# Autodesk Inventor assembly: Assey-N-N-body
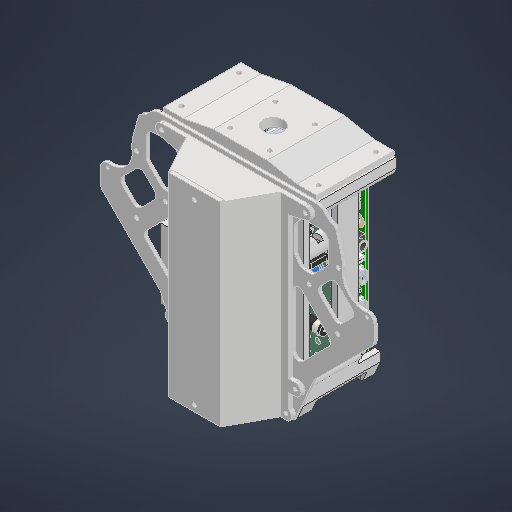
[picture p0: Inventor's stored thumbnail of the model, 512x512]
Saved by Autodesk Inventor 2026 (Build 300175050, 175E)
## iProperties
Created: 2026-03-17
Part Number: Assey-N-N-body
Document SubType Name: Assembly
Designer: kamada
Author: kamada
## Documents named in this file (11)
- C:\Users\marim\ドキュメント\KiCad\Project\Nexus\Nexus-3dmodel\Assey-N-N-body.iam
- C:\Users\marim\ドキュメント\KiCad\Project\Nexus\Nexus-3dmodel\NewBody-back.ipt
- C:\Users\marim\ドキュメント\KiCad\Project\Nexus\Nexus-3dmodel\Nexus-pcb.iam
- C:\Users\marim\ドキュメント\KiCad\Project\Nexus\Nexus-3dmodel\N-NBody.ipt
- C:\Users\marim\ドキュメント\KiCad\Project\Nexus\Nexus-3dmodel\NewBody.ipt
- C:\Users\marim\ドキュメント\KiCad\Project\Nexus\Nexus-3dmodel\NNFront.ipt
- C:\Users\marim\ドキュメント\KiCad\Project\Nexus\Nexus-3dmodel\daiza.ipt
- C:\Users\marim\ドキュメント\KiCad\Project\Nexus\Nexus-3dmodel\WMR-433-BK.ipt
- C:\Users\marim\ドキュメント\KiCad\Project\Nexus\Nexus-3dmodel\NN-Ura.ipt
- C:\Users\marim\ドキュメント\KiCad\Project\Nexus\Nexus-3dmodel\3sLiPo.ipt
- C:\Users\marim\ドキュメント\KiCad\Project\Nexus\Nexus-3dmodel\ff-hta.ipt
## Components (10 placed, 10 different names)
1. NewBody-back:1 — メイト:5, メイト:6, メイト:7, メイト:8, メイト:15, メイト:16, フラッシュ:3, フラッシュ:4, フラッシュ:5, メイト:29, フラッシュ:6, フラッシュ:7, フラッシュ:8
2. Nexus-pcb:1 [sub-assembly] — メイト:1, メイト:2, メイト:3, メイト:4, メイト:15, メイト:16
3. N-NBody:1 — フラッシュ:3, フラッシュ:4, フラッシュ:5, メイト:18, メイト:19, メイト:26, メイト:27, メイト:28
4. NewBody:1 — メイト:18, メイト:19, メイト:22, メイト:34, メイト:35, フラッシュ:9, フラッシュ:10
5. NNFront:1 — メイト:22, フラッシュ:9, フラッシュ:10, フラッシュ:11
6. daiza:1 — メイト:26, メイト:27, メイト:28
7. WMR-433-BK:1 — メイト:29, メイト:30, 角度:1
8. NN-Ura:1 — フラッシュ:6, フラッシュ:7, フラッシュ:8
9. 3sLiPo:1 — メイト:32, 角度:2, メイト:34, メイト:35, メイト:36, 角度:3
10. ff-hta:1 — フラッシュ:11
## Relationships (40: Mate 26, Flush 9, Angle 3, Symmetry 2)
- メイト:1 [Mate]: Nexus-pcb:1
- メイト:2 [Mate]: Nexus-pcb:1
- メイト:3 [Mate]: Nexus-pcb:1
- メイト:4 [Mate]: Nexus-pcb:1
- 対称度:1 [Symmetry]
- メイト:5 [Mate]: NewBody-back:1
- メイト:6 [Mate]: NewBody-back:1
- メイト:7 [Mate]: NewBody-back:1
- メイト:8 [Mate]: NewBody-back:1
- 対称度:2 [Symmetry]
- メイト:9 [Mate]
- メイト:14 [Mate]
- メイト:15 [Mate] (3 mm): NewBody-back:1 ↔ Nexus-pcb:1
- メイト:16 [Mate] (1 mm): NewBody-back:1 ↔ Nexus-pcb:1
- フラッシュ:3 [Flush]: NewBody-back:1 ↔ N-NBody:1
- フラッシュ:4 [Flush]: NewBody-back:1 ↔ N-NBody:1
- フラッシュ:5 [Flush]: NewBody-back:1 ↔ N-NBody:1
- メイト:18 [Mate]: N-NBody:1 ↔ NewBody:1
- メイト:19 [Mate]: N-NBody:1 ↔ NewBody:1
- メイト:22 [Mate]: NewBody:1 ↔ NNFront:1
- メイト:26 [Mate]: N-NBody:1 ↔ daiza:1
- メイト:27 [Mate]: N-NBody:1 ↔ daiza:1
- メイト:28 [Mate]: N-NBody:1 ↔ daiza:1
- メイト:29 [Mate]: NewBody-back:1 ↔ WMR-433-BK:1
- メイト:30 [Mate]: WMR-433-BK:1
- 角度:1 [Angle] (0 deg): WMR-433-BK:1
- メイト:31 [Mate]
- フラッシュ:6 [Flush]: NewBody-back:1 ↔ NN-Ura:1
- フラッシュ:7 [Flush]: NewBody-back:1 ↔ NN-Ura:1
- フラッシュ:8 [Flush]: NewBody-back:1 ↔ NN-Ura:1
- メイト:32 [Mate]: 3sLiPo:1
- 角度:2 [Angle] (0 deg): 3sLiPo:1
- メイト:33 [Mate]
- メイト:34 [Mate] (0.2 mm): NewBody:1 ↔ 3sLiPo:1
- メイト:35 [Mate]: NewBody:1 ↔ 3sLiPo:1
- フラッシュ:9 [Flush]: NewBody:1 ↔ NNFront:1
- メイト:36 [Mate]: 3sLiPo:1
- 角度:3 [Angle] (0 deg): 3sLiPo:1
- フラッシュ:10 [Flush]: NewBody:1 ↔ NNFront:1
- フラッシュ:11 [Flush]: NNFront:1 ↔ ff-hta:1
